# Autodesk Inventor assembly: Nut Assmbly
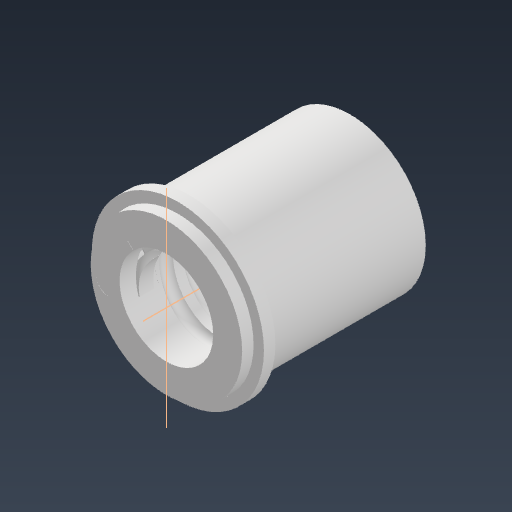
[picture p0: Inventor's stored thumbnail of the model, 512x512]
Saved by Autodesk Inventor 2021 (Build 250183000, 183)
## iProperties
Created: 2020-10-14
Part Number: Nut Assmbly
Document SubType Name: Assembly
Designer: Eugene Tang
Mass: 913.167 g
Surface Area: 1337.58 cm^2
Volume: 913.167 cm^3
Density: 1 g/cm^3
Author: Eugene Tang
## Documents named in this file (4)
- C:\Users\teuge\OneDrive - Curtin University of Technology Australia\Y4S2\DFM\Group Project\CAD\Parts\Nut Assmbly.iam
- C:\Users\teuge\OneDrive - Curtin University of Technology Australia\Y4S2\DFM\Group Project\CAD\Parts\Front Returd Mech.ipt
- C:\Users\teuge\OneDrive - Curtin University of Technology Australia\Y4S2\DFM\Group Project\CAD\Parts\Nut.ipt
- C:\Users\teuge\OneDrive - Curtin University of Technology Australia\Y4S2\DFM\Group Project\CAD\Parts\Rear Return Mech.ipt
## Components (3 placed, 3 different names)
1. Front Returd Mech:1 — Mate:1, Mate:2, Mate:3
2. Nut:1 — Mate:1, Mate:2, Mate:3, Mate:5, Mate:6, Mate:7
3. Rear Return Mech:1 — Mate:5, Mate:6, Mate:7
## Relationships (6: Mate 6)
- Mate:1: Front Returd Mech:1 ↔ Nut:1
- Mate:2: Front Returd Mech:1 ↔ Nut:1
- Mate:3: Front Returd Mech:1 ↔ Nut:1
- Mate:5: Nut:1 ↔ Rear Return Mech:1
- Mate:6: Nut:1 ↔ Rear Return Mech:1
- Mate:7: Nut:1 ↔ Rear Return Mech:1
